# Autodesk Inventor assembly: PÁRA-CHOQUE TRASEIRO
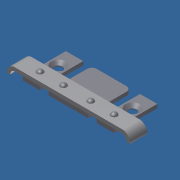
[picture p0: Inventor's stored thumbnail of the model, 180x180]
Saved by Autodesk Inventor 2012 SP1 (Build 160190100, 190)
## iProperties
Created: 2012-07-23
Part Number: PÁRA-CHOQUE TRASEIRO
Document SubType Name: Assembly
Designer: bruno.silveira
Author: bruno.silveira
## Documents named in this file (6)
- F:\CAMINHÃO-BITONEIRA-(SENAI)\PÁRA-CHOQUE TRASEIRO\PÁRA-CHOQUE TRASEIRO.iam
- F:\CAMINHÃO-BITONEIRA-(SENAI)\PÁRA-CHOQUE TRASEIRO\PLACA(45).ipt
- F:\CAMINHÃO-BITONEIRA-(SENAI)\PÁRA-CHOQUE TRASEIRO\LAMINA(46).ipt
- F:\CAMINHÃO-BITONEIRA-(SENAI)\PÁRA-CHOQUE TRASEIRO\SUPORTE(44).ipt
- F:\CAMINHÃO-BITONEIRA-(SENAI)\PÁRA-CHOQUE TRASEIRO\DIN 661 - A 3 x 10 x 6.ipt
- F:\CAMINHÃO-BITONEIRA-(SENAI)\PÁRA-CHOQUE TRASEIRO\DIN 660 - A 3 x 12 x 6.ipt
## Components (8 placed, 5 different names)
1. PLACA(45):1 — Mate:1, Mate:2, Mate:3
2. LAMINA(46):1 — Mate:1, Mate:2, Mate:3, Mate:4, Mate:5, Mate:6, Mate:7, Flush:1, Flush:2, Mate:8, Mate:9, Mate:12, Mate:13
3. SUPORTE(44):1 — Mate:4, Mate:5, Flush:2
4. SUPORTE(44):2 — Mate:6, Mate:7, Flush:1
5. DIN 660 - A 3 x 12 x 6:1 — Mate:12, Mate:13
6. DIN 660 - A 3 x 12 x 6:2
7. DIN 661 - A 3 x 10 x 6:1 — Mate:8, Mate:9
8. DIN 661 - A 3 x 10 x 6:2
## Component patterns: (2 elements, first: DIN 660 - A 3 x 12 x 6:1), (2 elements, first: DIN 661 - A 3 x 10 x 6:1)
## Relationships (13: Mate 11, Flush 2)
- Mate:1: PLACA(45):1 ↔ LAMINA(46):1
- Mate:2: PLACA(45):1 ↔ LAMINA(46):1
- Mate:3: PLACA(45):1 ↔ LAMINA(46):1
- Mate:4: LAMINA(46):1 ↔ SUPORTE(44):1
- Mate:5: LAMINA(46):1 ↔ SUPORTE(44):1
- Mate:6: LAMINA(46):1 ↔ SUPORTE(44):2
- Mate:7: LAMINA(46):1 ↔ SUPORTE(44):2
- Flush:1: LAMINA(46):1 ↔ SUPORTE(44):2
- Flush:2: LAMINA(46):1 ↔ SUPORTE(44):1
- Mate:8: LAMINA(46):1 ↔ DIN 661 - A 3 x 10 x 6:1
- Mate:9: LAMINA(46):1 ↔ DIN 661 - A 3 x 10 x 6:1
- Mate:12: LAMINA(46):1 ↔ DIN 660 - A 3 x 12 x 6:1
- Mate:13: LAMINA(46):1 ↔ DIN 660 - A 3 x 12 x 6:1
